# Autodesk Inventor assembly: TWambat Side Frame
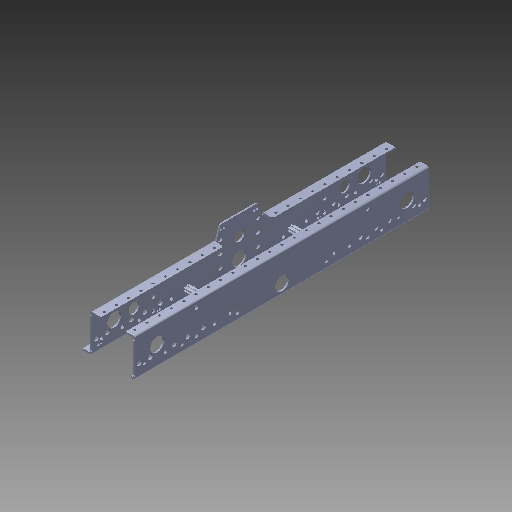
[picture p0: Inventor's stored thumbnail of the model, 512x512]
Saved by Autodesk Inventor 2019 (Build 230136000, 136)
## iProperties
Created: 2019-12-10
Part Number: TWambat Side Frame
Document SubType Name: Assembly
Designer: james
Author: james
## Documents named in this file (4)
- F:\JimsRobot\FIRSTRobots\Design\TWambat\TWambat Side Frame.iam
- F:\JimsRobot\FIRSTRobots\Design\TWambat\TWambat Inside Sheet.ipt
- F:\JimsRobot\FIRSTRobots\Design\Library\AndyMark\Churro 3375.ipt
- F:\JimsRobot\FIRSTRobots\Design\TWambat\TWambat Outside Sheet.ipt
## Components (4 placed, 3 different names)
1. TWambat Inside Sheet:1 — Mate:1, Mate:2, Mate:3, Mate:4
2. Churro 3375:1 — Mate:1, Mate:2, Mate:5, Mate:6
3. Churro 3375:2 — Mate:3, Mate:4, Mate:7
4. TWambat Outside Sheet:1 — Mate:5, Mate:6, Mate:7
## Relationships (7: Mate 7)
- Mate:1: TWambat Inside Sheet:1 ↔ Churro 3375:1
- Mate:2: TWambat Inside Sheet:1 ↔ Churro 3375:1
- Mate:3: TWambat Inside Sheet:1 ↔ Churro 3375:2
- Mate:4: TWambat Inside Sheet:1 ↔ Churro 3375:2
- Mate:5: Churro 3375:1 ↔ TWambat Outside Sheet:1
- Mate:6: Churro 3375:1 ↔ TWambat Outside Sheet:1
- Mate:7: Churro 3375:2 ↔ TWambat Outside Sheet:1
